# Autodesk Inventor assembly: Palma
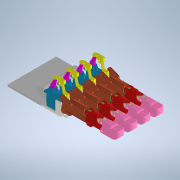
[picture p0: Inventor's stored thumbnail of the model, 180x180]
Saved by Autodesk Inventor 2020.4 (Build 244396010, 396A)
## iProperties
Created: 2021-08-20
Part Number: Palma
Document SubType Name: Assembly
Designer: chalo
Author: chalo
## Documents named in this file (4)
- C:\Users\chalo\OneDrive\Documents\GitHub\Interfaces-Biomedicas-2021\Gonzalo Palarea\Inventor\_completa\Palma.iam
- C:\Users\chalo\OneDrive\Documents\GitHub\Interfaces-Biomedicas-2021\Gonzalo Palarea\Inventor\tipo2\Prototipo2.iam
- C:\Users\chalo\OneDrive\Documents\GitHub\Interfaces-Biomedicas-2021\Gonzalo Palarea\Inventor\tipo2\Palma.ipt
- C:\Users\chalo\OneDrive\Documents\GitHub\Interfaces-Biomedicas-2021\Gonzalo Palarea\Inventor\referencias\18650.ipt
## Components (6 placed, 3 different names)
1. Prototipo2:1 [sub-assembly] — Flush:1, Flush:2, Flush:3, Mate:1, Flush:4
2. Prototipo2:2 [sub-assembly] — Flush:1, Mate:1, Mate:2, Flush:4, Flush:5, Flush:7
3. Prototipo2:3 [sub-assembly] — Flush:2, Mate:2, Mate:3, Flush:5, Flush:6
4. Prototipo2:4 [sub-assembly] — Flush:3, Mate:3, Flush:6
5. Palma:1 — Flush:7
6. 18650:2
## Relationships (10: Flush 7, Mate 3)
- Flush:1: Prototipo2:1 ↔ Prototipo2:2
- Flush:2: Prototipo2:1 ↔ Prototipo2:3
- Flush:3: Prototipo2:1 ↔ Prototipo2:4
- Mate:1 (7 mm): Prototipo2:1 ↔ Prototipo2:2
- Mate:2 (7 mm): Prototipo2:2 ↔ Prototipo2:3
- Mate:3 (7 mm): Prototipo2:3 ↔ Prototipo2:4
- Flush:4: Prototipo2:1 ↔ Prototipo2:2
- Flush:5: Prototipo2:2 ↔ Prototipo2:3
- Flush:6: Prototipo2:3 ↔ Prototipo2:4
- Flush:7: Prototipo2:2 ↔ Palma:1
